# Autodesk Inventor assembly: RoboArm Assembly 1
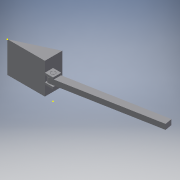
[picture p0: Inventor's stored thumbnail of the model, 180x180]
Saved by Autodesk Inventor 2019 (Build 230136000, 136)
## iProperties
Created: 2020-02-03
Part Number: RoboArm Assembly 1
Document SubType Name: Assembly
Designer: mbird
Author: mbird
## Documents named in this file (4)
- C:\Users\mbird\OneDrive\Documents\Inventor\digger\RoboArm Assembly 1.iam
- C:\Users\mbird\OneDrive\Documents\Inventor\digger\RoboArm 2020 scoop.ipt
- C:\Users\mbird\OneDrive\Documents\Inventor\digger\RoboArm 2020 Arm.ipt
- C:\Users\mbird\OneDrive\Documents\Inventor\digger\RoboArm 2020 Rod.ipt
## Components (3 placed, 3 different names)
1. RoboArm 2020 scoop:1 — Mate:1, Mate:3, Mate:4
2. RoboArm 2020 Arm:1 — Mate:2, Mate:3
3. RoboArm 2020 Rod:1 — Mate:1, Mate:2, Mate:4
## Relationships (4: Mate 4)
- Mate:1: RoboArm 2020 scoop:1 ↔ RoboArm 2020 Rod:1
- Mate:2: RoboArm 2020 Arm:1 ↔ RoboArm 2020 Rod:1
- Mate:3 (2.5 mm): RoboArm 2020 scoop:1 ↔ RoboArm 2020 Arm:1
- Mate:4: RoboArm 2020 scoop:1 ↔ RoboArm 2020 Rod:1
